# Autodesk Inventor assembly: POM_T5_09
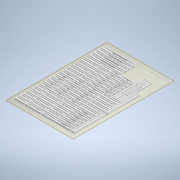
[picture p0: Inventor's stored thumbnail of the model, 180x180]
Saved by Autodesk Inventor 2020 (Build 240168000, 168)
## iProperties
Created: 2021-08-27
Part Number: POM_T5_09
Document SubType Name: Assembly
Designer: Masato
Author: Masato
## Documents named in this file (17)
- C:\Inventor\SUSTAINA-OP\Cam\POM_T5_09.iam
- C:\Inventor\SUSTAINA-OP\Cam\DisposableBoard.ipt
- C:\Inventor\SUSTAINA-OP\Jig\BackLink_diagonal_Jig.ipt
- C:\Inventor\SUSTAINA-OP\Jig\Cockpit_back_frame_Jig.ipt
- C:\Inventor\SUSTAINA-OP\Jig\Cockpit_battery_back_door_Jig.ipt
- C:\Inventor\SUSTAINA-OP\Jig\Cockpit_battery_front_frame_Jig.ipt
- C:\Inventor\SUSTAINA-OP\Jig\Cockpit_carrier_board_frame_Jig.ipt
- C:\Inventor\SUSTAINA-OP\Jig\Cockpit_circuit_board_frame_Jig.ipt
- C:\Inventor\SUSTAINA-OP\Jig\Foot_root_block_Jig.ipt
- C:\Inventor\SUSTAINA-OP\Jig\FrontLink_diagonal_Jig.ipt
- C:\Inventor\SUSTAINA-OP\Jig\Head_horn_frame_Jig.ipt
- C:\Inventor\SUSTAINA-OP\Jig\Leg_joint_yaw_frame_Jig.ipt
- C:\Inventor\SUSTAINA-OP\Jig\Shoulder_horn_frame_Jig.ipt
- C:\Inventor\SUSTAINA-OP\Jig\Trunk_chest_frame_Jig_1.ipt
- C:\Inventor\SUSTAINA-OP\Jig\Trunk_chest_frame_Jig_2.ipt
- C:\Inventor\SUSTAINA-OP\Jig\Trunk_lower_side_frame_Jig.ipt
- C:\Inventor\SUSTAINA-OP\Jig\UpperArm_diagonal_Jig.ipt
## Components (82 placed, 16 different names)
1. DisposableBoard:1 — メイト:2, メイト:1, フラッシュ:1, フラッシュ:2, メイト:4, フラッシュ:3, フラッシュ:4, メイト:5, メイト:7, メイト:9, メイト:11, メイト:13, メイト:15, メイト:17, メイト:19, メイト:20, メイト:21, メイト:22, メイト:27, メイト:28, メイト:37
2. Cockpit_back_frame_Jig:1
3. BackLink_diagonal_Jig:1 — メイト:4, フラッシュ:3, フラッシュ:4, フラッシュ:5, メイト:6, フラッシュ:12, フラッシュ:16, フラッシュ:17
4. BackLink_diagonal_Jig:2
5. BackLink_diagonal_Jig:3
6. BackLink_diagonal_Jig:4
7. BackLink_diagonal_Jig:5
8. BackLink_diagonal_Jig:6 — フラッシュ:8, メイト:12
9. Cockpit_battery_back_door_Jig:1 — メイト:5, フラッシュ:5, メイト:6, フラッシュ:6, メイト:8
10. Cockpit_battery_front_frame_Jig:1 — メイト:7, フラッシュ:6, メイト:8, フラッシュ:7, メイト:10
11. Cockpit_battery_back_door_Jig:2
12. Cockpit_battery_front_frame_Jig:2
13. Cockpit_battery_back_door_Jig:3
14. Cockpit_battery_front_frame_Jig:3
15. Cockpit_battery_back_door_Jig:4
16. Cockpit_battery_front_frame_Jig:4
17. Cockpit_battery_back_door_Jig:5
18. Cockpit_battery_front_frame_Jig:5
19. Cockpit_battery_back_door_Jig:6
20. Cockpit_battery_front_frame_Jig:6
21. Trunk_chest_frame_Jig_2:1 — メイト:9, フラッシュ:7, メイト:10
22. Trunk_chest_frame_Jig_2:2
23. Trunk_chest_frame_Jig_2:3
24. Trunk_chest_frame_Jig_2:4
25. Trunk_chest_frame_Jig_2:5
26. Trunk_chest_frame_Jig_2:6 — メイト:30
27. Head_horn_frame_Jig:1 — メイト:13, フラッシュ:9, メイト:14, メイト:16
28. Head_horn_frame_Jig:2
29. Head_horn_frame_Jig:3
30. Head_horn_frame_Jig:4
31. Head_horn_frame_Jig:5
32. Head_horn_frame_Jig:6 — メイト:32
33. Shoulder_horn_frame_Jig:1 — メイト:11, フラッシュ:8, メイト:12, フラッシュ:9, メイト:14, フラッシュ:10
34. Trunk_lower_side_frame_Jig:1 — メイト:15, フラッシュ:10, メイト:16, メイト:18
35. FrontLink_diagonal_Jig:1 — メイト:17, メイト:18, メイト:30, メイト:36
36. Shoulder_horn_frame_Jig:2
37. Trunk_lower_side_frame_Jig:2
38. FrontLink_diagonal_Jig:2
39. Shoulder_horn_frame_Jig:3
40. Trunk_lower_side_frame_Jig:3
41. FrontLink_diagonal_Jig:3
42. Shoulder_horn_frame_Jig:4
43. Trunk_lower_side_frame_Jig:4
44. FrontLink_diagonal_Jig:4
45. Shoulder_horn_frame_Jig:5
46. Trunk_lower_side_frame_Jig:5
47. FrontLink_diagonal_Jig:5
48. Shoulder_horn_frame_Jig:6 — メイト:31
49. Trunk_lower_side_frame_Jig:6 — メイト:33
50. FrontLink_diagonal_Jig:6 — メイト:34, メイト:38
51. Trunk_chest_frame_Jig_1:1 — メイト:19, フラッシュ:12, メイト:24, メイト:31
52. UpperArm_diagonal_Jig:1 — メイト:21, メイト:26, メイト:34
53. Trunk_chest_frame_Jig_1:2
54. UpperArm_diagonal_Jig:2
55. Trunk_chest_frame_Jig_1:3
56. UpperArm_diagonal_Jig:3
57. Trunk_chest_frame_Jig_1:4
58. UpperArm_diagonal_Jig:4
59. Trunk_chest_frame_Jig_1:5
60. UpperArm_diagonal_Jig:5
61. Trunk_chest_frame_Jig_1:6 — メイト:35
62. UpperArm_diagonal_Jig:6
63. Leg_joint_yaw_frame_Jig:1 — メイト:20, メイト:24, メイト:25, メイト:32
64. Foot_root_block_Jig:1 — メイト:22, メイト:25, メイト:26, メイト:33
65. Leg_joint_yaw_frame_Jig:2
66. Foot_root_block_Jig:2
67. Leg_joint_yaw_frame_Jig:3
68. Foot_root_block_Jig:3
69. Leg_joint_yaw_frame_Jig:4
70. Foot_root_block_Jig:4
71. Leg_joint_yaw_frame_Jig:5
72. Foot_root_block_Jig:5
73. Leg_joint_yaw_frame_Jig:6
74. Foot_root_block_Jig:6
75. Cockpit_carrier_board_frame_Jig:1 — メイト:27, フラッシュ:16, メイト:35
76. Cockpit_carrier_board_frame_Jig:2
77. Cockpit_carrier_board_frame_Jig:3
78. Cockpit_carrier_board_frame_Jig:4
79. Cockpit_circuit_board_frame_Jig:1 — メイト:28, メイト:36, フラッシュ:17
80. Cockpit_circuit_board_frame_Jig:2 — メイト:39
81. Cockpit_carrier_board_frame_Jig:5 — メイト:37, メイト:38, メイト:39
82. Cockpit_carrier_board_frame_Jig:6
## Component patterns: (6 elements, first: BackLink_diagonal_Jig:1), (6 elements, first: Cockpit_battery_back_door_Jig:1 + Cockpit_battery_front_frame_Jig:1), (6 elements, first: Trunk_chest_frame_Jig_2:1), (6 elements, first: Head_horn_frame_Jig:1), (6 elements, first: Shoulder_horn_frame_Jig:1 + Trunk_lower_side_frame_Jig:1 + FrontLink_diagonal_Jig:1), (6 elements, first: Trunk_chest_frame_Jig_1:1 + UpperArm_diagonal_Jig:1), (6 elements, first: Leg_joint_yaw_frame_Jig:1 + Foot_root_block_Jig:1), (4 elements, first: Cockpit_carrier_board_frame_Jig:1), (2 elements, first: Cockpit_circuit_board_frame_Jig:1), (2 elements, first: Cockpit_carrier_board_frame_Jig:5)
## Relationships (49: Mate 36, Flush 13)
- メイト:2 [Mate]: DisposableBoard:1
- メイト:1 [Mate]: DisposableBoard:1
- フラッシュ:1 [Flush]: DisposableBoard:1
- フラッシュ:2 [Flush]: DisposableBoard:1
- メイト:4 [Mate]: DisposableBoard:1 ↔ BackLink_diagonal_Jig:1
- フラッシュ:3 [Flush] (1.5 mm): DisposableBoard:1 ↔ BackLink_diagonal_Jig:1
- フラッシュ:4 [Flush] (1.5 mm): DisposableBoard:1 ↔ BackLink_diagonal_Jig:1
- メイト:5 [Mate]: DisposableBoard:1 ↔ Cockpit_battery_back_door_Jig:1
- フラッシュ:5 [Flush]: BackLink_diagonal_Jig:1 ↔ Cockpit_battery_back_door_Jig:1
- メイト:6 [Mate] (2.5 mm): BackLink_diagonal_Jig:1 ↔ Cockpit_battery_back_door_Jig:1
- メイト:7 [Mate]: DisposableBoard:1 ↔ Cockpit_battery_front_frame_Jig:1
- フラッシュ:6 [Flush]: Cockpit_battery_back_door_Jig:1 ↔ Cockpit_battery_front_frame_Jig:1
- メイト:8 [Mate] (2.5 mm): Cockpit_battery_back_door_Jig:1 ↔ Cockpit_battery_front_frame_Jig:1
- メイト:9 [Mate]: DisposableBoard:1 ↔ Trunk_chest_frame_Jig_2:1
- フラッシュ:7 [Flush]: Cockpit_battery_front_frame_Jig:1 ↔ Trunk_chest_frame_Jig_2:1
- メイト:10 [Mate] (2.5 mm): Cockpit_battery_front_frame_Jig:1 ↔ Trunk_chest_frame_Jig_2:1
- メイト:11 [Mate]: DisposableBoard:1 ↔ Shoulder_horn_frame_Jig:1
- フラッシュ:8 [Flush]: BackLink_diagonal_Jig:6 ↔ Shoulder_horn_frame_Jig:1
- メイト:12 [Mate] (2.5 mm): BackLink_diagonal_Jig:6 ↔ Shoulder_horn_frame_Jig:1
- メイト:13 [Mate]: DisposableBoard:1 ↔ Head_horn_frame_Jig:1
- フラッシュ:9 [Flush]: Head_horn_frame_Jig:1 ↔ Shoulder_horn_frame_Jig:1
- メイト:14 [Mate] (2.5 mm): Head_horn_frame_Jig:1 ↔ Shoulder_horn_frame_Jig:1
- メイト:15 [Mate]: DisposableBoard:1 ↔ Trunk_lower_side_frame_Jig:1
- フラッシュ:10 [Flush]: Shoulder_horn_frame_Jig:1 ↔ Trunk_lower_side_frame_Jig:1
- メイト:16 [Mate] (2.5 mm): Head_horn_frame_Jig:1 ↔ Trunk_lower_side_frame_Jig:1
- メイト:17 [Mate]: DisposableBoard:1 ↔ FrontLink_diagonal_Jig:1
- メイト:18 [Mate] (2.5 mm): Trunk_lower_side_frame_Jig:1 ↔ FrontLink_diagonal_Jig:1
- メイト:19 [Mate]: DisposableBoard:1 ↔ Trunk_chest_frame_Jig_1:1
- メイト:20 [Mate]: DisposableBoard:1 ↔ Leg_joint_yaw_frame_Jig:1
- メイト:21 [Mate]: DisposableBoard:1 ↔ UpperArm_diagonal_Jig:1
- メイト:22 [Mate]: DisposableBoard:1 ↔ Foot_root_block_Jig:1
- フラッシュ:12 [Flush]: BackLink_diagonal_Jig:1 ↔ Trunk_chest_frame_Jig_1:1
- メイト:24 [Mate] (2.5 mm): Trunk_chest_frame_Jig_1:1 ↔ Leg_joint_yaw_frame_Jig:1
- メイト:25 [Mate] (2.5 mm): Leg_joint_yaw_frame_Jig:1 ↔ Foot_root_block_Jig:1
- メイト:26 [Mate] (2.5 mm): UpperArm_diagonal_Jig:1 ↔ Foot_root_block_Jig:1
- メイト:27 [Mate]: DisposableBoard:1 ↔ Cockpit_carrier_board_frame_Jig:1
- メイト:28 [Mate]: DisposableBoard:1 ↔ Cockpit_circuit_board_frame_Jig:1
- フラッシュ:16 [Flush]: BackLink_diagonal_Jig:1 ↔ Cockpit_carrier_board_frame_Jig:1
- メイト:30 [Mate] (2.5 mm): Trunk_chest_frame_Jig_2:6 ↔ FrontLink_diagonal_Jig:1
- メイト:31 [Mate] (2.5 mm): Shoulder_horn_frame_Jig:6 ↔ Trunk_chest_frame_Jig_1:1
- メイト:32 [Mate] (2.5 mm): Head_horn_frame_Jig:6 ↔ Leg_joint_yaw_frame_Jig:1
- メイト:33 [Mate] (2.5 mm): Trunk_lower_side_frame_Jig:6 ↔ Foot_root_block_Jig:1
- メイト:34 [Mate] (2.5 mm): FrontLink_diagonal_Jig:6 ↔ UpperArm_diagonal_Jig:1
- メイト:35 [Mate] (2.5 mm): Trunk_chest_frame_Jig_1:6 ↔ Cockpit_carrier_board_frame_Jig:1
- メイト:36 [Mate] (2.5 mm): FrontLink_diagonal_Jig:1 ↔ Cockpit_circuit_board_frame_Jig:1
- フラッシュ:17 [Flush]: BackLink_diagonal_Jig:1 ↔ Cockpit_circuit_board_frame_Jig:1
- メイト:37 [Mate]: DisposableBoard:1 ↔ Cockpit_carrier_board_frame_Jig:5
- メイト:38 [Mate] (2.5 mm): FrontLink_diagonal_Jig:6 ↔ Cockpit_carrier_board_frame_Jig:5
- メイト:39 [Mate] (2.5 mm): Cockpit_circuit_board_frame_Jig:2 ↔ Cockpit_carrier_board_frame_Jig:5
